# Autodesk Inventor assembly: GlidelejrehusAssembly
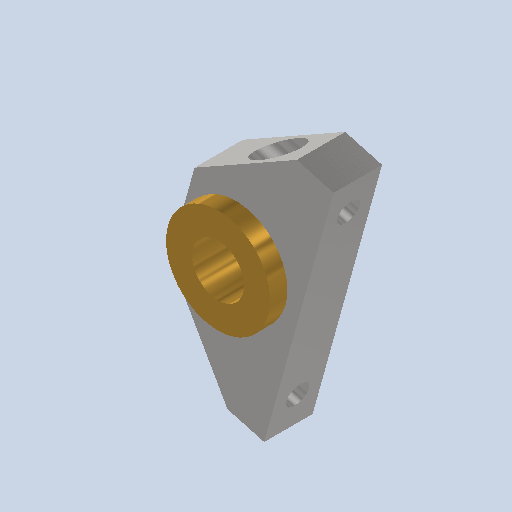
[picture p0: Inventor's stored thumbnail of the model, 512x512]
Saved by Autodesk Inventor 2022.2 (Build 262287000, 287)
## iProperties
Created: 2022-04-19
Part Number: GlidelejrehusAssembly
Document SubType Name: Assembly
Designer: Finn Oriwohl
Author: Finn Oriwohl
## Documents named in this file (3)
- H:\inventor ting\Mekatronik beercart git\Beercart CAD\Workspaces\Workspace\beercart assembly - mekatronik\Frame\GlidelejrehusAssembly.iam
- H:\inventor ting\Mekatronik beercart git\Beercart CAD\Workspaces\Workspace\Build drawings\Glidelejrehus.ipt
- H:\inventor ting\Mekatronik beercart git\Beercart CAD\Workspaces\Workspace\Build drawings\glide lejre bushing.ipt
## Components (2 placed, 2 different names)
1. Glidelejrehus:1
2. glide lejre bushing:1
## Relationships (2: Flush 1, Insert 1)
- [Flush]: Glidelejrehus:1 ↔ glide lejre bushing:1
- [Insert]: Glidelejrehus:1 ↔ glide lejre bushing:1
